# Autodesk Inventor assembly: Final Assembly
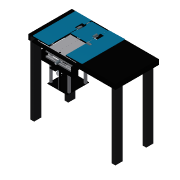
[picture p0: Inventor's stored thumbnail of the model, 180x180]
Saved by Autodesk Inventor 2016 (Build 200138000, 138)
## iProperties
Created: 2016-04-10
Part Number: Final Assembly
Document SubType Name: Assembly
Designer: Andrea
Author: Andrea
## Documents named in this file (10)
- C:\Users\Ariana\Downloads\Capstone CAD\Capstone CAD\Final Assembly.iam
- C:\Users\Ariana\Downloads\Capstone CAD\Capstone CAD\Mid Flap System Assembly.iam
- C:\Users\Ariana\Downloads\Capstone CAD\Capstone CAD\Table Top and Flaps.iam
- C:\Users\Ariana\Downloads\Capstone CAD\Capstone CAD\Motor + Attachment\Motor and Bracket.iam
- C:\Users\Ariana\Downloads\Capstone CAD\Capstone CAD\Motor + Attachment\Motor and Bracket_MIR.iam
- C:\Users\Ariana\Downloads\Capstone CAD\Capstone CAD\Table Frame Side.ipt
- C:\Users\Ariana\Downloads\Capstone CAD\Capstone CAD\Table Frame Back.ipt
- C:\Users\Ariana\Downloads\Capstone CAD\Capstone CAD\Table Frame Front.ipt
- C:\Users\Ariana\Downloads\Capstone CAD\Capstone CAD\Table Leg.ipt
- C:\Users\Ariana\Downloads\Capstone CAD\Capstone CAD\Delivery\Delivery.iam
## Components (14 placed, 9 different names)
1. Table Top and Flaps:1 [sub-assembly] — Mate:1, Mate:2, Mate:3, Mate:4, Angle:1, Mate:5, Mate:8, Mate:9, Mate:10, Mate:11, Mate:12, Flush:2, Flush:3, Mate:14, Mate:15, Mate:16, Mate:17, Mate:18, Flush:4, Flush:5, Flush:6, Mate:21, Mate:22, Mate:29, Mate:30, Flush:8
2. Mid Flap System Assembly:1 [sub-assembly] — Mate:4, Angle:1, Flush:2, Flush:3
3. Motor and Bracket:1 [sub-assembly] — Mate:8, Mate:9, Mate:10
4. Motor and Bracket_MIR:1 [sub-assembly] — Mate:5, Mate:13
5. Motor and Bracket:2 [sub-assembly] — Mate:11, Mate:12, Mate:13
6. Table Frame Side:1 — Mate:16, Mate:17, Mate:19, Flush:7, Mate:25
7. Table Frame Side:2 — Mate:14, Mate:15, Mate:20, Mate:23, Mate:27
8. Table Frame Back:1 — Mate:18, Flush:4, Mate:19, Mate:24, Mate:26
9. Table Frame Front:1 — Flush:5, Mate:20, Flush:6, Mate:21, Mate:28
10. Table Leg:1 — Flush:7, Mate:22
11. Table Leg:2 — Mate:23, Mate:24
12. Table Leg:3 — Mate:25, Mate:26
13. Table Leg:4 — Mate:27, Mate:28
14. Delivery:1 [sub-assembly] — Mate:29, Mate:30, Flush:8
## Relationships (36: Mate 28, Flush 7, Angle 1)
- Mate:1: Table Top and Flaps:1
- Mate:2: Table Top and Flaps:1
- Mate:3: Table Top and Flaps:1
- Mate:4: Table Top and Flaps:1 ↔ Mid Flap System Assembly:1
- Angle:1 (0 deg): Table Top and Flaps:1 ↔ Mid Flap System Assembly:1
- Mate:5: Table Top and Flaps:1 ↔ Motor and Bracket_MIR:1
- Mate:8: Table Top and Flaps:1 ↔ Motor and Bracket:1
- Mate:9 (2.54 mm): Table Top and Flaps:1 ↔ Motor and Bracket:1
- Mate:10 (11.8364 mm): Table Top and Flaps:1 ↔ Motor and Bracket:1
- Mate:11: Table Top and Flaps:1 ↔ Motor and Bracket:2
- Mate:12 (2.54 mm): Table Top and Flaps:1 ↔ Motor and Bracket:2
- Mate:13 (87.2744 mm): Motor and Bracket_MIR:1 ↔ Motor and Bracket:2
- Flush:2: Table Top and Flaps:1 ↔ Mid Flap System Assembly:1
- Flush:3 (101.6 mm): Table Top and Flaps:1 ↔ Mid Flap System Assembly:1
- Mate:14: Table Top and Flaps:1 ↔ Table Frame Side:2
- Mate:15: Table Top and Flaps:1 ↔ Table Frame Side:2
- Mate:16: Table Top and Flaps:1 ↔ Table Frame Side:1
- Mate:17: Table Top and Flaps:1 ↔ Table Frame Side:1
- Mate:18: Table Top and Flaps:1 ↔ Table Frame Back:1
- Flush:4: Table Top and Flaps:1 ↔ Table Frame Back:1
- Mate:19: Table Frame Side:1 ↔ Table Frame Back:1
- Flush:5: Table Top and Flaps:1 ↔ Table Frame Front:1
- Mate:20: Table Frame Side:2 ↔ Table Frame Front:1
- Flush:6: Table Top and Flaps:1 ↔ Table Frame Front:1
- Mate:21: Table Top and Flaps:1 ↔ Table Frame Front:1
- Flush:7: Table Frame Side:1 ↔ Table Leg:1
- Mate:22: Table Top and Flaps:1 ↔ Table Leg:1
- Mate:23: Table Frame Side:2 ↔ Table Leg:2
- Mate:24: Table Frame Back:1 ↔ Table Leg:2
- Mate:25: Table Frame Side:1 ↔ Table Leg:3
- Mate:26: Table Frame Back:1 ↔ Table Leg:3
- Mate:27: Table Frame Side:2 ↔ Table Leg:4
- Mate:28: Table Frame Front:1 ↔ Table Leg:4
- Mate:29: Table Top and Flaps:1 ↔ Delivery:1
- Mate:30: Table Top and Flaps:1 ↔ Delivery:1
- Flush:8: Table Top and Flaps:1 ↔ Delivery:1
